# Autodesk Inventor assembly: Assembly
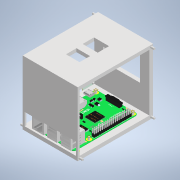
[picture p0: Inventor's stored thumbnail of the model, 180x180]
Saved by Autodesk Inventor 2021 (Build 250183000, 183)
## iProperties
Created: 2020-04-05
Part Number: Assembly
Document SubType Name: Assembly
Designer: Daniel
Author: Daniel
## Documents named in this file (3)
- E:\Program Files\Autodesk\parts\Assembly.iam
- E:\Program Files\Autodesk\parts\weather_base.ipt
- E:\Program Files\Autodesk\parts\Raspberry Pi Model B.ipt
## Components (2 placed, 2 different names)
1. weather_base:1 — Mate:1, Mate:2
2. Raspberry Pi Model B:1 — Mate:1, Mate:2
## Relationships (2: Mate 2)
- Mate:1: weather_base:1 ↔ Raspberry Pi Model B:1
- Mate:2: weather_base:1 ↔ Raspberry Pi Model B:1
